# Autodesk Inventor assembly: Drive-A Unit
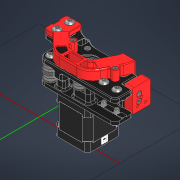
[picture p0: Inventor's stored thumbnail of the model, 180x180]
Saved by Autodesk Inventor 2022.2 (Build 262287010, 287A)
## iProperties
Created: 2022-03-14
Part Number: Drive-A Unit
Document SubType Name: Assembly
Designer: sleib
Author: sleib
## Documents named in this file (18)
- C:\Users\sleib\Projekte\Voron-2\CAD\Inventor\Drive-A Unit.iam
- C:\Users\sleib\Projekte\Voron-2\CAD\Inventor\Drive-A Frame.ipt
- C:\Users\sleib\Projekte\Voron-2\CAD\Inventor\NEMA17 Black.ipt
- C:\Users\sleib\Projekte\Voron-2\CAD\Inventor\GT2 16T Pulley (6mm).ipt
- C:\Users\sleib\Projekte\Voron-2\CAD\Inventor\M3x30 SHCS.ipt
- C:\Users\sleib\Projekte\Voron-2\CAD\Inventor\Z Belt-Clamp Upper.ipt
- C:\Users\sleib\Projekte\Voron-2\CAD\Inventor\M5x16 BHCS.ipt
- C:\Users\sleib\Projekte\Voron-2\CAD\Inventor\M5x10 BHCS.ipt
- C:\Users\sleib\Projekte\Voron-2\CAD\Inventor\M5x30 BHCS.ipt
- C:\Users\sleib\Projekte\Voron-2\CAD\Inventor\M5 Spacer (1mm).ipt
- C:\Users\sleib\Projekte\Voron-2\CAD\Inventor\Bearing F695-ZZ.ipt
- C:\Users\sleib\Projekte\Voron-2\CAD\Inventor\Cable-Cover Drive-A.ipt
- C:\Users\sleib\Projekte\Voron-2\CAD\Inventor\M3x12 SHCS.ipt
- C:\Users\sleib\Projekte\Voron-2\CAD\Inventor\M3 Threaded Insert.ipt
- C:\Users\sleib\Projekte\Voron-2\CAD\Inventor\Chain Retainer-Bracket.ipt
- C:\Users\sleib\Projekte\Voron-2\CAD\Inventor\M3 Hexnut.ipt
- C:\Users\sleib\Projekte\Voron-2\CAD\Inventor\Chain Adapter.ipt
- C:\Users\sleib\Projekte\Voron-2\CAD\Inventor\M3x16 SHCS.ipt
## Components (41 placed, 17 different names)
1. Drive-A Frame:1 — Fluchtend:1, Passend:5, Passend:6, Passend:7, Passend:11, Passend:12, Passend:13, Passend:14, Passend:17, Passend:18, Passend:21, Passend:22, Passend:23, Passend:24, Passend:25, Passend:26, Passend:27, Passend:28, Passend:29, Passend:30, Passend:31, Passend:47, Passend:48, Passend:56, Passend:57, Passend:62, Passend:63, Fluchtend:3, Fluchtend:4, Passend:66, Passend:71, Passend:72, Passend:73, Winkel:3, Passend:85, Passend:86
2. NEMA17 Black:1 — Passend:4, Fluchtend:2, Passend:8, Passend:9, Passend:10, Passend:14
3. GT2 16T Pulley (6mm):1 — Passend:4, Fluchtend:2
4. M3x30 SHCS:1 — Passend:5, Passend:9, Passend:12
5. M3x30 SHCS:2 — Passend:6, Passend:8, Passend:11
6. M3x30 SHCS:3 — Passend:7, Passend:10, Passend:13
7. Z Belt-Clamp Upper:1 — Passend:15, Passend:16, Passend:19, Passend:20, Passend:21
8. M5x16 BHCS:1 — Passend:15, Passend:17, Passend:19
9. M5x16 BHCS:2 — Passend:16, Passend:18, Passend:20
10. M5x10 BHCS:1 — Passend:22, Passend:28
11. M5x10 BHCS:2 — Passend:23, Passend:29
12. M5x10 BHCS:3 — Passend:24, Passend:26
13. M5x10 BHCS:4 — Passend:25, Passend:27
14. M5x30 BHCS:1 — Passend:30, Passend:32, Passend:33, Passend:34, Passend:35, Passend:36, Passend:37, Passend:38, Passend:39, Passend:48
15. M5x30 BHCS:2 — Passend:31, Passend:49, Passend:50, Passend:51, Passend:52, Passend:56
16. M5 Spacer (1mm):1 — Passend:32, Passend:40
17. M5 Spacer (1mm):2 — Passend:35, Passend:42, Passend:43
18. M5 Spacer (1mm):3 — Passend:36, Passend:43, Passend:46
19. M5 Spacer (1mm):4 — Passend:39, Passend:44, Passend:47
20. M5 Spacer (1mm):5 — Passend:49, Passend:53
21. M5 Spacer (1mm):6 — Passend:52, Passend:54, Passend:57
22. Bearing F695-ZZ:1 — Passend:33, Passend:40, Passend:41
23. Bearing F695-ZZ:2 — Passend:34, Passend:41, Passend:42
24. Bearing F695-ZZ:3 — Passend:37, Passend:45, Passend:46
25. Bearing F695-ZZ:4 — Passend:38, Passend:44, Passend:45
26. Bearing F695-ZZ:5 — Passend:50, Passend:53, Passend:55
27. Bearing F695-ZZ:6 — Passend:51, Passend:54, Passend:55
28. Cable-Cover Drive-A:1 — Passend:58, Passend:59, Passend:60, Passend:61, Passend:66
29. M3x12 SHCS:1 — Passend:58, Passend:60, Passend:65
30. M3x12 SHCS:2 — Passend:59, Passend:61, Passend:64
31. M3 Threaded Insert:1 — Passend:62, Fluchtend:3, Passend:64
32. M3 Threaded Insert:2 — Passend:63, Fluchtend:4, Passend:65
33. Chain Retainer-Bracket:1 — Passend:69, Passend:70, Passend:71, Passend:88, Passend:89
34. M3 Hexnut:1 — Passend:69, Passend:74, Passend:75, Passend:83, Passend:88
35. M3 Hexnut:2 — Passend:70, Passend:74, Passend:75, Passend:84, Passend:89
36. Chain Adapter:1 — Passend:76, Passend:77, Passend:78, Fluchtend:5, Fluchtend:6, Fluchtend:7, Passend:79, Passend:80, Passend:81, Passend:82, Passend:85, Passend:86, Fluchtend:8
37. M3 Threaded Insert:3 — Passend:78, Fluchtend:5
38. M3 Threaded Insert:4 — Passend:77, Fluchtend:6
39. M3 Threaded Insert:5 — Passend:76, Fluchtend:7
40. M3x16 SHCS:1 — Passend:79, Passend:81, Passend:83
41. M3x16 SHCS:2 — Passend:80, Passend:82, Passend:84
## Relationships (92: Mate 83, Flush 8, Angle 1)
- Fluchtend:1 [Flush]: Drive-A Frame:1
- Passend:4 [Mate]: NEMA17 Black:1 ↔ GT2 16T Pulley (6mm):1
- Fluchtend:2 [Flush]: NEMA17 Black:1 ↔ GT2 16T Pulley (6mm):1
- Passend:5 [Mate]: Drive-A Frame:1 ↔ M3x30 SHCS:1
- Passend:6 [Mate]: Drive-A Frame:1 ↔ M3x30 SHCS:2
- Passend:7 [Mate]: Drive-A Frame:1 ↔ M3x30 SHCS:3
- Passend:8 [Mate]: NEMA17 Black:1 ↔ M3x30 SHCS:2
- Passend:9 [Mate]: NEMA17 Black:1 ↔ M3x30 SHCS:1
- Passend:10 [Mate]: NEMA17 Black:1 ↔ M3x30 SHCS:3
- Passend:11 [Mate]: Drive-A Frame:1 ↔ M3x30 SHCS:2
- Passend:12 [Mate]: Drive-A Frame:1 ↔ M3x30 SHCS:1
- Passend:13 [Mate]: Drive-A Frame:1 ↔ M3x30 SHCS:3
- Passend:14 [Mate]: Drive-A Frame:1 ↔ NEMA17 Black:1
- Passend:15 [Mate]: Z Belt-Clamp Upper:1 ↔ M5x16 BHCS:1
- Passend:16 [Mate]: Z Belt-Clamp Upper:1 ↔ M5x16 BHCS:2
- Passend:17 [Mate]: Drive-A Frame:1 ↔ M5x16 BHCS:1
- Passend:18 [Mate]: Drive-A Frame:1 ↔ M5x16 BHCS:2
- Passend:19 [Mate]: Z Belt-Clamp Upper:1 ↔ M5x16 BHCS:1
- Passend:20 [Mate]: Z Belt-Clamp Upper:1 ↔ M5x16 BHCS:2
- Passend:21 [Mate]: Drive-A Frame:1 ↔ Z Belt-Clamp Upper:1
- Passend:22 [Mate]: Drive-A Frame:1 ↔ M5x10 BHCS:1
- Passend:23 [Mate]: Drive-A Frame:1 ↔ M5x10 BHCS:2
- Passend:24 [Mate]: Drive-A Frame:1 ↔ M5x10 BHCS:3
- Passend:25 [Mate]: Drive-A Frame:1 ↔ M5x10 BHCS:4
- Passend:26 [Mate]: Drive-A Frame:1 ↔ M5x10 BHCS:3
- Passend:27 [Mate]: Drive-A Frame:1 ↔ M5x10 BHCS:4
- Passend:28 [Mate]: Drive-A Frame:1 ↔ M5x10 BHCS:1
- Passend:29 [Mate]: Drive-A Frame:1 ↔ M5x10 BHCS:2
- Passend:30 [Mate]: Drive-A Frame:1 ↔ M5x30 BHCS:1
- Passend:31 [Mate]: Drive-A Frame:1 ↔ M5x30 BHCS:2
- Passend:32 [Mate]: M5x30 BHCS:1 ↔ M5 Spacer (1mm):1
- Passend:33 [Mate]: M5x30 BHCS:1 ↔ Bearing F695-ZZ:1
- Passend:34 [Mate]: M5x30 BHCS:1 ↔ Bearing F695-ZZ:2
- Passend:35 [Mate]: M5x30 BHCS:1 ↔ M5 Spacer (1mm):2
- Passend:36 [Mate]: M5x30 BHCS:1 ↔ M5 Spacer (1mm):3
- Passend:37 [Mate]: M5x30 BHCS:1 ↔ Bearing F695-ZZ:3
- Passend:38 [Mate]: M5x30 BHCS:1 ↔ Bearing F695-ZZ:4
- Passend:39 [Mate]: M5x30 BHCS:1 ↔ M5 Spacer (1mm):4
- Passend:40 [Mate]: M5 Spacer (1mm):1 ↔ Bearing F695-ZZ:1
- Passend:41 [Mate]: Bearing F695-ZZ:1 ↔ Bearing F695-ZZ:2
- Passend:42 [Mate]: M5 Spacer (1mm):2 ↔ Bearing F695-ZZ:2
- Passend:43 [Mate]: M5 Spacer (1mm):2 ↔ M5 Spacer (1mm):3
- Passend:44 [Mate]: M5 Spacer (1mm):4 ↔ Bearing F695-ZZ:4
- Passend:45 [Mate]: Bearing F695-ZZ:3 ↔ Bearing F695-ZZ:4
- Passend:46 [Mate]: M5 Spacer (1mm):3 ↔ Bearing F695-ZZ:3
- Passend:47 [Mate]: Drive-A Frame:1 ↔ M5 Spacer (1mm):4
- Passend:48 [Mate]: Drive-A Frame:1 ↔ M5x30 BHCS:1
- Passend:49 [Mate]: M5x30 BHCS:2 ↔ M5 Spacer (1mm):5
- Passend:50 [Mate]: M5x30 BHCS:2 ↔ Bearing F695-ZZ:5
- Passend:51 [Mate]: M5x30 BHCS:2 ↔ Bearing F695-ZZ:6
- Passend:52 [Mate]: M5x30 BHCS:2 ↔ M5 Spacer (1mm):6
- Passend:53 [Mate]: M5 Spacer (1mm):5 ↔ Bearing F695-ZZ:5
- Passend:54 [Mate]: M5 Spacer (1mm):6 ↔ Bearing F695-ZZ:6
- Passend:55 [Mate]: Bearing F695-ZZ:5 ↔ Bearing F695-ZZ:6
- Passend:56 [Mate]: Drive-A Frame:1 ↔ M5x30 BHCS:2
- Passend:57 [Mate]: Drive-A Frame:1 ↔ M5 Spacer (1mm):6
- Passend:58 [Mate]: Cable-Cover Drive-A:1 ↔ M3x12 SHCS:1
- Passend:59 [Mate]: Cable-Cover Drive-A:1 ↔ M3x12 SHCS:2
- Passend:60 [Mate]: Cable-Cover Drive-A:1 ↔ M3x12 SHCS:1
- Passend:61 [Mate]: Cable-Cover Drive-A:1 ↔ M3x12 SHCS:2
- Passend:62 [Mate]: Drive-A Frame:1 ↔ M3 Threaded Insert:1
- Passend:63 [Mate]: Drive-A Frame:1 ↔ M3 Threaded Insert:2
- Fluchtend:3 [Flush]: Drive-A Frame:1 ↔ M3 Threaded Insert:1
- Fluchtend:4 [Flush]: Drive-A Frame:1 ↔ M3 Threaded Insert:2
- Passend:64 [Mate]: M3x12 SHCS:2 ↔ M3 Threaded Insert:1
- Passend:65 [Mate]: M3x12 SHCS:1 ↔ M3 Threaded Insert:2
- Passend:66 [Mate]: Drive-A Frame:1 ↔ Cable-Cover Drive-A:1
- Passend:69 [Mate]: Chain Retainer-Bracket:1 ↔ M3 Hexnut:1
- Passend:70 [Mate]: Chain Retainer-Bracket:1 ↔ M3 Hexnut:2
- Passend:71 [Mate]: Drive-A Frame:1 ↔ Chain Retainer-Bracket:1
- Passend:72 [Mate]: Drive-A Frame:1
- Passend:73 [Mate]: Drive-A Frame:1
- Winkel:3 [Angle] (0 deg): Drive-A Frame:1
- Passend:74 [Mate]: M3 Hexnut:1 ↔ M3 Hexnut:2
- Passend:75 [Mate] (8 mm): M3 Hexnut:1 ↔ M3 Hexnut:2
- Passend:76 [Mate]: Chain Adapter:1 ↔ M3 Threaded Insert:5
- Passend:77 [Mate]: Chain Adapter:1 ↔ M3 Threaded Insert:4
- Passend:78 [Mate]: Chain Adapter:1 ↔ M3 Threaded Insert:3
- Fluchtend:5 [Flush]: Chain Adapter:1 ↔ M3 Threaded Insert:3
- Fluchtend:6 [Flush]: Chain Adapter:1 ↔ M3 Threaded Insert:4
- Fluchtend:7 [Flush]: Chain Adapter:1 ↔ M3 Threaded Insert:5
- Passend:79 [Mate]: Chain Adapter:1 ↔ M3x16 SHCS:1
- Passend:80 [Mate]: Chain Adapter:1 ↔ M3x16 SHCS:2
- Passend:81 [Mate]: Chain Adapter:1 ↔ M3x16 SHCS:1
- Passend:82 [Mate]: Chain Adapter:1 ↔ M3x16 SHCS:2
- Passend:83 [Mate]: M3 Hexnut:1 ↔ M3x16 SHCS:1
- Passend:84 [Mate]: M3 Hexnut:2 ↔ M3x16 SHCS:2
- Passend:85 [Mate]: Drive-A Frame:1 ↔ Chain Adapter:1
- Passend:86 [Mate] (2 mm): Drive-A Frame:1 ↔ Chain Adapter:1
- Passend:88 [Mate] (0.115 mm): Chain Retainer-Bracket:1 ↔ M3 Hexnut:1
- Passend:89 [Mate] (0.116 mm): Chain Retainer-Bracket:1 ↔ M3 Hexnut:2
- Fluchtend:8 [Flush] (0.11 mm): Chain Adapter:1
